# Autodesk Inventor assembly: FTC ROBOT DRIVE TRAIN
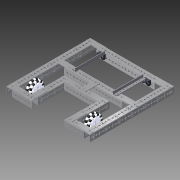
[picture p0: Inventor's stored thumbnail of the model, 180x180]
Saved by Autodesk Inventor 2015 (Build 190159000, 159)
## iProperties
Created: 2014-10-06
Part Number: FTC ROBOT DRIVE TRAIN
Document SubType Name: Assembly
Designer: lethcoec
Author: lethcoec
## Documents named in this file (10)
- H:\FTC Cascade effect\FTC ROBOT DRIVE TRAIN.iam
- H:\Channel288mm.ipt
- \\st-svr\studenthdrives$\18\LethcoeC\FTC Cascade effect\Imported Components\Channel160mm\Channel160mm.ipt
- \\st-svr\studenthdrives$\18\LethcoeC\FTC Cascade effect\Imported Components\Channel96mm\Channel96mm.ipt
- \\st-svr\studenthdrives$\18\LethcoeC\FTC Cascade effect\FTC Parts\Subassemblies\Bracket and Screws.iam
- H:\Inventor\Channel416mm.ipt
- \\st-svr\studenthdrives$\18\LethcoeC\FTC Cascade effect\Imported Components\BracketFlat\BracketFlat.ipt
- \\st-svr\studenthdrives$\18\LethcoeC\FTC Cascade effect\FTC Parts\Subassemblies\Dual Omni Wheel.iam
- \\st-svr\studenthdrives$\18\LethcoeC\FTC Cascade effect\Imported Components\LMax\LMax.ipt
- \\st-svr\studenthdrives$\18\LethcoeC\FTC Cascade effect\L Bracket with holes.ipt
## Components (26 placed, 9 different names)
1. Channel288mm:1 — Mate:62, Mate:64, Mate:67, Mate:76, Mate:77, Mate:101, Mate:104
2. Channel160mm:1 — Mate:9, Flush:17, Flush:18, Mate:11, Flush:21, Flush:22, Mate:53, Mate:54, Mate:55
3. Channel160mm:3 — Mate:10, Flush:19, Flush:20, Flush:23, Mate:43, Mate:48, Mate:49
4. Channel96mm:1 — Mate:9, Flush:17, Flush:18, Mate:56, Mate:58, Mate:80, Flush:24
5. Channel96mm:2 — Mate:10, Flush:19, Flush:20, Mate:44, Mate:45, Mate:46, Mate:71, Mate:72
6. Channel160mm:5 — Mate:11, Flush:21, Flush:22, Flush:23, Mate:50, Mate:51, Mate:52, Mate:74, Mate:75
7. Channel288mm:6 — Mate:61, Mate:70, Mate:82, Mate:90, Mate:91, Mate:97, Mate:98
8. Bracket and Screws:1 [sub-assembly] — Mate:45, Mate:46, Mate:73
9. Bracket and Screws:2 [sub-assembly] — Mate:48, Mate:49, Mate:50
10. Bracket and Screws:3 [sub-assembly] — Mate:43, Mate:44
11. Bracket and Screws:4 [sub-assembly] — Mate:54, Mate:55
12. Bracket and Screws:5 [sub-assembly] — Mate:56, Mate:58, Mate:81
13. Bracket and Screws:6 [sub-assembly] — Mate:61, Mate:85, Flush:25
14. Bracket and Screws:7 [sub-assembly] — Mate:51, Mate:52, Mate:53
15. Bracket and Screws:8 [sub-assembly] — Mate:67
16. Bracket and Screws:9 [sub-assembly] — Mate:62, Mate:64, Mate:83, Mate:84
17. Bracket and Screws:10 [sub-assembly] — Mate:70, Mate:78, Mate:79, Mate:82
18. Channel416mm:1 — Mate:80, Mate:81, Flush:24, Mate:83, Mate:84, Mate:85, Mate:86, Mate:87
19. Channel416mm:2 — Mate:71, Mate:72, Mate:73, Mate:78, Mate:79, Mate:88, Mate:89
20. BracketFlat:1 — Mate:74, Mate:75, Mate:76, Mate:77
21. Dual Omni Wheel:1 [sub-assembly] — Mate:86, Mate:87
22. Dual Omni Wheel:2 [sub-assembly] — Mate:88, Mate:89
23. LMax:1 — Mate:90, Mate:91, Flush:25, Mate:102, Mate:103
24. LMax:3 — Mate:97, Mate:98, Mate:99, Mate:100
25. L Bracket with holes:1 — Mate:99, Mate:100, Mate:101
26. L Bracket with holes:2 — Mate:102, Mate:103, Mate:104
## Relationships (60: Mate 51, Flush 9)
- Mate:9: Channel160mm:1 ↔ Channel96mm:1
- Flush:17: Channel160mm:1 ↔ Channel96mm:1
- Flush:18: Channel160mm:1 ↔ Channel96mm:1
- Mate:10: Channel160mm:3 ↔ Channel96mm:2
- Flush:19: Channel160mm:3 ↔ Channel96mm:2
- Flush:20: Channel160mm:3 ↔ Channel96mm:2
- Mate:11: Channel160mm:1 ↔ Channel160mm:5
- Flush:21: Channel160mm:1 ↔ Channel160mm:5
- Flush:22: Channel160mm:1 ↔ Channel160mm:5
- Flush:23: Channel160mm:3 ↔ Channel160mm:5
- Mate:43: Channel160mm:3 ↔ Bracket and Screws:3
- Mate:44: Channel96mm:2 ↔ Bracket and Screws:3
- Mate:45: Channel96mm:2 ↔ Bracket and Screws:1
- Mate:46: Channel96mm:2 ↔ Bracket and Screws:1
- Mate:48: Channel160mm:3 ↔ Bracket and Screws:2
- Mate:49: Channel160mm:3 ↔ Bracket and Screws:2
- Mate:50: Channel160mm:5 ↔ Bracket and Screws:2
- Mate:51: Channel160mm:5 ↔ Bracket and Screws:7
- Mate:52: Channel160mm:5 ↔ Bracket and Screws:7
- Mate:53: Channel160mm:1 ↔ Bracket and Screws:7
- Mate:54: Channel160mm:1 ↔ Bracket and Screws:4
- Mate:55: Channel160mm:1 ↔ Bracket and Screws:4
- Mate:56: Channel96mm:1 ↔ Bracket and Screws:5
- Mate:58: Channel96mm:1 ↔ Bracket and Screws:5
- Mate:61: Channel288mm:6 ↔ Bracket and Screws:6
- Mate:62: Channel288mm:1 ↔ Bracket and Screws:9
- Mate:64: Channel288mm:1 ↔ Bracket and Screws:9
- Mate:67: Channel288mm:1 ↔ Bracket and Screws:8
- Mate:70: Channel288mm:6 ↔ Bracket and Screws:10
- Mate:71: Channel96mm:2 ↔ Channel416mm:2
- Mate:72: Channel96mm:2 ↔ Channel416mm:2
- Mate:73: Bracket and Screws:1 ↔ Channel416mm:2
- Mate:74: Channel160mm:5 ↔ BracketFlat:1
- Mate:75: Channel160mm:5 ↔ BracketFlat:1
- Mate:76: Channel288mm:1 ↔ BracketFlat:1
- Mate:77: Channel288mm:1 ↔ BracketFlat:1
- Mate:78: Bracket and Screws:10 ↔ Channel416mm:2
- Mate:79: Bracket and Screws:10 ↔ Channel416mm:2
- Mate:80: Channel96mm:1 ↔ Channel416mm:1
- Mate:81: Bracket and Screws:5 ↔ Channel416mm:1
- Flush:24: Channel96mm:1 ↔ Channel416mm:1
- Mate:82: Channel288mm:6 ↔ Bracket and Screws:10
- Mate:83: Bracket and Screws:9 ↔ Channel416mm:1
- Mate:84: Bracket and Screws:9 ↔ Channel416mm:1
- Mate:85: Bracket and Screws:6 ↔ Channel416mm:1
- Mate:86: Channel416mm:1 ↔ Dual Omni Wheel:1
- Mate:87: Channel416mm:1 ↔ Dual Omni Wheel:1
- Mate:88: Channel416mm:2 ↔ Dual Omni Wheel:2
- Mate:89: Channel416mm:2 ↔ Dual Omni Wheel:2
- Mate:90: Channel288mm:6 ↔ LMax:1
- Mate:91: Channel288mm:6 ↔ LMax:1
- Flush:25: Bracket and Screws:6 ↔ LMax:1
- Mate:97: Channel288mm:6 ↔ LMax:3
- Mate:98: Channel288mm:6 ↔ LMax:3
- Mate:99: LMax:3 ↔ L Bracket with holes:1
- Mate:100: LMax:3 ↔ L Bracket with holes:1
- Mate:101: Channel288mm:1 ↔ L Bracket with holes:1
- Mate:102: LMax:1 ↔ L Bracket with holes:2
- Mate:103: LMax:1 ↔ L Bracket with holes:2
- Mate:104: Channel288mm:1 ↔ L Bracket with holes:2
